# Autodesk Inventor assembly: Batteriepack
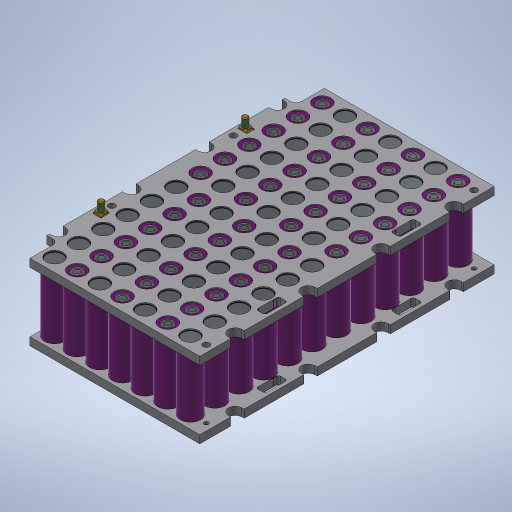
[picture p0: Inventor's stored thumbnail of the model, 512x512]
Saved by Autodesk Inventor 2024 (Build 280153000, 153)
## iProperties
Created: 2025-03-26
Part Number: Batteriepack
Document SubType Name: Assembly
Designer: David Lill
Author: David Lill
## Documents named in this file (5)
- C:\Users\Angela Ogrenda\Documents\Backup Inventor\Batteriepack.iam
- C:\Users\Angela Ogrenda\Documents\Backup Inventor\Platte1.ipt
- C:\Users\Angela Ogrenda\Documents\Backup Inventor\18650.ipt
- C:\Users\Angela Ogrenda\Documents\Backup Inventor\REDCUBEM7x7.ipt
- C:\Users\Angela Ogrenda\Documents\Backup Inventor\Abstandhalter.ipt
## Components (90 placed, 4 different names)
1. Platte1:3 — Einfügen:5, Einfügen:6, Einfügen:7, Einfügen:8
2. Platte1:4 — Einfügen:9, Einfügen:10, Einfügen:11, Einfügen:12
3. REDCUBEM7x7:1
4. REDCUBEM7x7:2
5. Abstandhalter:1 — Einfügen:12
6. Abstandhalter:2 — Einfügen:11
7. 18650:1 — Einfügen:5
8. 18650:4 — Einfügen:8
9. 18650:5
10. 18650:6
11. 18650:7
12. 18650:8
13. 18650:9
14. 18650:10
15. 18650:11
16. 18650:12
17. 18650:13
18. 18650:14 — Einfügen:10
19. 18650:25
20. 18650:26
21. 18650:27
22. 18650:28
23. 18650:29
24. 18650:30
25. 18650:31
26. 18650:32
27. 18650:33
28. 18650:34
29. 18650:35
30. 18650:36
31. 18650:37
32. 18650:38
33. 18650:39
34. 18650:40
35. 18650:41
36. 18650:42
37. 18650:43
38. 18650:44
39. 18650:45
40. 18650:46
41. 18650:47
42. 18650:48
43. 18650:49 — Einfügen:9
44. 18650:50
45. 18650:51
46. 18650:52
47. 18650:53
48. 18650:54
49. 18650:55
50. 18650:56
51. 18650:57
52. 18650:58
53. 18650:59
54. 18650:60
55. 18650:2 — Einfügen:7
56. 18650:3 — Einfügen:6
57. 18650:15
58. 18650:16
59. 18650:17
60. 18650:18
61. 18650:19
62. 18650:20
63. 18650:21
64. 18650:22
65. 18650:23
66. 18650:24
67. 18650:61
68. 18650:62
69. 18650:63
70. 18650:64
71. 18650:65
72. 18650:66
73. 18650:67
74. 18650:68
75. 18650:69
76. 18650:70
77. 18650:71
78. 18650:72
79. 18650:73
80. 18650:74
81. 18650:75
82. 18650:76
83. 18650:77
84. 18650:78
85. 18650:79
86. 18650:80
87. 18650:81
88. 18650:82
89. 18650:83
90. 18650:84
## Component patterns: (4 elements), (3 elements), (6 elements, first: 18650:1 + 18650:4), Komponentenanordnung 5:2 (6 elements), Komponentenanordnung 5:3 (6 elements), Komponentenanordnung 5:4 (6 elements), (6 elements, first: 18650:2 + 18650:3), Komponentenanordnung 6:2 (6 elements), Komponentenanordnung 6:3 (6 elements)
## Relationships (8: Insert 8)
- Einfügen:5 [Insert]: Platte1:3 ↔ 18650:1
- Einfügen:6 [Insert]: Platte1:3 ↔ 18650:3
- Einfügen:7 [Insert]: Platte1:3 ↔ 18650:2
- Einfügen:8 [Insert]: Platte1:3 ↔ 18650:4
- Einfügen:9 [Insert]: Platte1:4 ↔ 18650:49
- Einfügen:10 [Insert]: Platte1:4 ↔ 18650:14
- Einfügen:11 [Insert]: Platte1:4 ↔ Abstandhalter:2
- Einfügen:12 [Insert]: Platte1:4 ↔ Abstandhalter:1
